# Autodesk Inventor assembly: Mecanum_Assembly
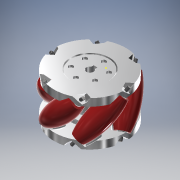
[picture p0: Inventor's stored thumbnail of the model, 180x180]
Saved by Autodesk Inventor 2018 (Build 220112000, 112)
## iProperties
Created: 2017-09-05
Part Number: Mecanum_Assembly
Document SubType Name: Assembly
Designer: P136265
Author: P136265
## Documents named in this file (8)
- C:\Users\P136265\Documents\mecanum-cad\Mecanum_Assembly.iam
- C:\Users\P136265\Documents\mecanum-cad\roller 8-19-6 bearing.ipt
- C:\Users\P136265\Documents\Inventor\Content Center Files\R2018\en-US\DIN 625 SKF(4)\DIN 625 SKF - SKF 619_8-2Z.ipt
- C:\Users\P136265\Documents\mecanum-cad\MecanumShaft.ipt
- C:\Users\P136265\Documents\mecanum-cad\PE_Sleeve.ipt
- C:\Users\P136265\Documents\mecanum-cad\CheekPlate.ipt
- C:\Users\P136265\Documents\mecanum-cad\MecanumHub.ipt
- C:\Users\P136265\Documents\mecanum-cad\Washer.ipt
## Components (45 placed, 7 different names)
1. CheekPlate:1 — Mate:11, Mate:12, Mate:13, Angle:3, Mate:18, Mate:19
2. CheekPlate:2 — Angle:3, Mate:14, Mate:15
3. MecanumHub:1 — Mate:18, Mate:19
4. roller 8-19-6 bearing:1 — Mate:1, Angle:1, Mate:2, Mate:3, Mate:4, Insert:1, Insert:2, Angle:2, Mate:9, Mate:15
5. MecanumShaft:1 — Angle:2, Mate:9, Mate:10
6. PE_Sleeve:1 — Mate:3, Mate:4
7. Washer:1 — Mate:5, Mate:6
8. Washer:2 — Mate:7, Mate:8, Mate:10
9. DIN 625 SKF- with two Z shields SKF 619/8-2Z:1 — Insert:1, Mate:7, Mate:8
10. DIN 625 SKF- with two Z shields SKF 619/8-2Z:2 — Insert:2, Mate:5, Mate:6
11. roller 8-19-6 bearing:2
12. MecanumShaft:2
13. PE_Sleeve:2
14. Washer:3
15. Washer:4
16. DIN 625 SKF- with two Z shields SKF 619/8-2Z:3
17. DIN 625 SKF- with two Z shields SKF 619/8-2Z:4
18. roller 8-19-6 bearing:3
19. MecanumShaft:3 — Mate:11
20. PE_Sleeve:3
21. Washer:5 — Mate:12
22. Washer:6
23. DIN 625 SKF- with two Z shields SKF 619/8-2Z:5
24. DIN 625 SKF- with two Z shields SKF 619/8-2Z:6
25. roller 8-19-6 bearing:4
26. MecanumShaft:4 — Mate:14
27. PE_Sleeve:4
28. Washer:7
29. Washer:8
30. DIN 625 SKF- with two Z shields SKF 619/8-2Z:7
31. DIN 625 SKF- with two Z shields SKF 619/8-2Z:8
32. roller 8-19-6 bearing:5 — Mate:13
33. MecanumShaft:5
34. PE_Sleeve:5
35. Washer:9
36. Washer:10
37. DIN 625 SKF- with two Z shields SKF 619/8-2Z:9
38. DIN 625 SKF- with two Z shields SKF 619/8-2Z:10
39. roller 8-19-6 bearing:6
40. MecanumShaft:6
41. PE_Sleeve:6
42. Washer:11
43. Washer:12
44. DIN 625 SKF- with two Z shields SKF 619/8-2Z:11
45. DIN 625 SKF- with two Z shields SKF 619/8-2Z:12
## Component patterns: (6 elements, first: roller 8-19-6 bearing:1 + MecanumShaft:1 + PE_Sleeve:1 + Washer:1 + Washer:2 + DIN 625 SKF- with two Z shields SKF 619/8-2Z:1 + DIN 625 SKF- with two Z shields SKF 619/8-2Z:2)
## Relationships (22: Mate 17, Angle 3, Insert 2)
- Mate:1 (75 mm): roller 8-19-6 bearing:1
- Angle:1 (45 deg): roller 8-19-6 bearing:1
- Mate:2: roller 8-19-6 bearing:1
- Mate:3: roller 8-19-6 bearing:1 ↔ PE_Sleeve:1
- Mate:4: roller 8-19-6 bearing:1 ↔ PE_Sleeve:1
- Insert:1: roller 8-19-6 bearing:1 ↔ DIN 625 SKF- with two Z shields SKF 619/8-2Z:1
- Insert:2: roller 8-19-6 bearing:1 ↔ DIN 625 SKF- with two Z shields SKF 619/8-2Z:2
- Mate:5: Washer:1 ↔ DIN 625 SKF- with two Z shields SKF 619/8-2Z:2
- Mate:6: Washer:1 ↔ DIN 625 SKF- with two Z shields SKF 619/8-2Z:2
- Mate:7: Washer:2 ↔ DIN 625 SKF- with two Z shields SKF 619/8-2Z:1
- Mate:8: Washer:2 ↔ DIN 625 SKF- with two Z shields SKF 619/8-2Z:1
- Angle:2 (0 deg): roller 8-19-6 bearing:1 ↔ MecanumShaft:1
- Mate:9: roller 8-19-6 bearing:1 ↔ MecanumShaft:1
- Mate:10 (18 mm): MecanumShaft:1 ↔ Washer:2
- Mate:11: CheekPlate:1 ↔ MecanumShaft:3
- Mate:12: CheekPlate:1 ↔ Washer:5
- Mate:13: CheekPlate:1 ↔ roller 8-19-6 bearing:5
- Angle:3 (0 deg): CheekPlate:1 ↔ CheekPlate:2
- Mate:14: CheekPlate:2 ↔ MecanumShaft:4
- Mate:15: CheekPlate:2 ↔ roller 8-19-6 bearing:1
- Mate:18: CheekPlate:1 ↔ MecanumHub:1
- Mate:19: CheekPlate:1 ↔ MecanumHub:1
